# Autodesk Inventor assembly: ISIS CubeSat STS PC104 Skeleton-MAR1
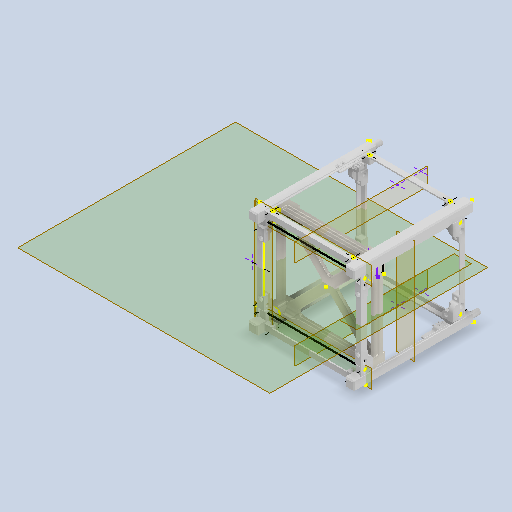
[picture p0: Inventor's stored thumbnail of the model, 512x512]
Saved by Autodesk Inventor 2023 (Build 270158000, 158)
## iProperties
Created: 2011-03-02
Part Number: ISIS CubeSat STS PC104 Skeleton-MAR1
Document SubType Name: Assembly
Designer: maylo
Sending System: PRO/ENGINEER BY PARAMETRIC TECHNOLOGY CORPORATION, 2003250
Preprocessor: PRO/ENGINEER BY PARAMETRIC TECHNOLOGY CORPORATION, 2003250
Title: 1U_STS_SKELETON
Revision Number: LAST_VERSION
## Documents named in this file (5)
- E:\Dropbox\AMSAT\Cube Sat Frame Info\ISIS\ISIS CubeSat STS PC104 Skeleton-MAR1.iam
- E:\Dropbox\AMSAT\Cube Sat Frame Info\ISIS\INTEGRATED_SIDE_FRAME_007B_ASM.iam
- E:\Dropbox\AMSAT\Cube Sat Frame Info\ISIS\REVE_02-1_ASSEMBLY_RIB_CDEF_ASM.iam
- E:\Dropbox\AMSAT\Cube Sat Frame Info\ISIS\SCREW_M2_5X6.ipt
- E:\Dropbox\AMSAT\CAD_backup_frequent_files_20200629\RT-IHU_heatsink STANDOFF-MAR1.ipt
## Components (5 placed, 5 different names)
1. INTEGRATED_SIDE_FRAME_007B_ASM_22 [sub-assembly] — Mate:4, Mate:5, Flush:3
2. INTEGRATED_SIDE_FRAME_007B_ASM_23 [sub-assembly] — Flush:2, Mate:2, Mate:3, Mate:8
3. REVE_02-1_ASSEMBLY_RIB_CDEF_ASM_32 [sub-assembly] — Flush:2, Mate:2, Mate:3, Mate:4, Mate:5, Flush:3, Mate:6, Mate:7, Flush:4
4. SCREW_M2_5X6:1 — Mate:6, Mate:7
5. RT-IHU_heatsink STANDOFF-MAR1:1 — Mate:8, Flush:4
## Relationships (10: Mate 7, Flush 3)
- Flush:2: INTEGRATED_SIDE_FRAME_007B_ASM_23 ↔ REVE_02-1_ASSEMBLY_RIB_CDEF_ASM_32
- Mate:2: INTEGRATED_SIDE_FRAME_007B_ASM_23 ↔ REVE_02-1_ASSEMBLY_RIB_CDEF_ASM_32
- Mate:3: INTEGRATED_SIDE_FRAME_007B_ASM_23 ↔ REVE_02-1_ASSEMBLY_RIB_CDEF_ASM_32
- Mate:4: INTEGRATED_SIDE_FRAME_007B_ASM_22 ↔ REVE_02-1_ASSEMBLY_RIB_CDEF_ASM_32
- Mate:5: INTEGRATED_SIDE_FRAME_007B_ASM_22 ↔ REVE_02-1_ASSEMBLY_RIB_CDEF_ASM_32
- Flush:3: INTEGRATED_SIDE_FRAME_007B_ASM_22 ↔ REVE_02-1_ASSEMBLY_RIB_CDEF_ASM_32
- Mate:6: REVE_02-1_ASSEMBLY_RIB_CDEF_ASM_32 ↔ SCREW_M2_5X6:1
- Mate:7: REVE_02-1_ASSEMBLY_RIB_CDEF_ASM_32 ↔ SCREW_M2_5X6:1
- Mate:8 (0.357 mm): INTEGRATED_SIDE_FRAME_007B_ASM_23 ↔ RT-IHU_heatsink STANDOFF-MAR1:1
- Flush:4: REVE_02-1_ASSEMBLY_RIB_CDEF_ASM_32 ↔ RT-IHU_heatsink STANDOFF-MAR1:1
